# Autodesk Inventor assembly: Gear Assembly
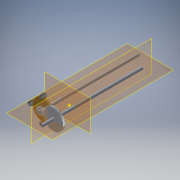
[picture p0: Inventor's stored thumbnail of the model, 180x180]
Saved by Autodesk Inventor 2016 (Build 200138000, 138)
## iProperties
Created: 2018-04-27
Part Number: Gear Assembly
Document SubType Name: Assembly
Designer: 2000083068
Author: 2000083068
## Documents named in this file (5)
- E:\Robotics\Off Season\Blannon\Gear Assembly.iam
- E:\Robotics\Off Season\Blannon\72t_Aluminum_Spur_Gear_20_DP_1_2_Hex_Bore_217-3576.ipt
- E:\Robotics\Off Season\Blannon\24t_Steel_Spur_Gear_20_DP_1_2_Hex_Bore_217-5464.ipt
- E:\Robotics\Off Season\Blannon\11t_Steel_Spur_Gear_20_DP_CIM_Motor_12t_Center_Distance_217-3107.ipt
- E:\Robotics\Off Season\Blannon\ThunderHex_Stock_18in.ipt
## Components (8 placed, 4 different names)
1. 72t_Aluminum_Spur_Gear_20_DP_1_2_Hex_Bore_217-3576:1 — Mate:1, Flush:1, Flush:2, Mate:6, Flush:4, Flush:5, Mate:12, Mate:15
2. 24t_Steel_Spur_Gear_20_DP_1_2_Hex_Bore_217-5464:1 — Mate:1, Flush:1, Flush:2, Mate:5, Mate:9, Mate:10, Mate:13
3. 72t_Aluminum_Spur_Gear_20_DP_1_2_Hex_Bore_217-3576:2 — Mate:7, Mate:8, Flush:3, Flush:4
4. 11t_Steel_Spur_Gear_20_DP_CIM_Motor_12t_Center_Distance_217-3107:1 — Mate:11, Flush:5
5. 11t_Steel_Spur_Gear_20_DP_CIM_Motor_12t_Center_Distance_217-3107:2 — Mate:5, Mate:6, Mate:14
6. 11t_Steel_Spur_Gear_20_DP_CIM_Motor_12t_Center_Distance_217-3107:3 — Mate:12, Mate:13
7. ThunderHex_Stock_18in:1 — Mate:7, Mate:8, Flush:3, Flush:6, Mate:16
8. ThunderHex_Stock_18in:2 — Mate:9, Mate:10, Mate:11, Flush:6
## Relationships (19: Mate 13, Flush 6)
- Mate:1: 72t_Aluminum_Spur_Gear_20_DP_1_2_Hex_Bore_217-3576:1 ↔ 24t_Steel_Spur_Gear_20_DP_1_2_Hex_Bore_217-5464:1
- Flush:1: 72t_Aluminum_Spur_Gear_20_DP_1_2_Hex_Bore_217-3576:1 ↔ 24t_Steel_Spur_Gear_20_DP_1_2_Hex_Bore_217-5464:1
- Flush:2: 72t_Aluminum_Spur_Gear_20_DP_1_2_Hex_Bore_217-3576:1 ↔ 24t_Steel_Spur_Gear_20_DP_1_2_Hex_Bore_217-5464:1
- Mate:5 (-42.164 mm): 24t_Steel_Spur_Gear_20_DP_1_2_Hex_Bore_217-5464:1 ↔ 11t_Steel_Spur_Gear_20_DP_CIM_Motor_12t_Center_Distance_217-3107:2
- Mate:6 (-12.7 mm): 72t_Aluminum_Spur_Gear_20_DP_1_2_Hex_Bore_217-3576:1 ↔ 11t_Steel_Spur_Gear_20_DP_CIM_Motor_12t_Center_Distance_217-3107:2
- Mate:7: 72t_Aluminum_Spur_Gear_20_DP_1_2_Hex_Bore_217-3576:2 ↔ ThunderHex_Stock_18in:1
- Mate:8: 72t_Aluminum_Spur_Gear_20_DP_1_2_Hex_Bore_217-3576:2 ↔ ThunderHex_Stock_18in:1
- Mate:9: 24t_Steel_Spur_Gear_20_DP_1_2_Hex_Bore_217-5464:1 ↔ ThunderHex_Stock_18in:2
- Mate:10: 24t_Steel_Spur_Gear_20_DP_1_2_Hex_Bore_217-5464:1 ↔ ThunderHex_Stock_18in:2
- Flush:3 (-50.8 mm): 72t_Aluminum_Spur_Gear_20_DP_1_2_Hex_Bore_217-3576:2 ↔ ThunderHex_Stock_18in:1
- Flush:4 (-12.7 mm): 72t_Aluminum_Spur_Gear_20_DP_1_2_Hex_Bore_217-3576:1 ↔ 72t_Aluminum_Spur_Gear_20_DP_1_2_Hex_Bore_217-3576:2
- Mate:11 (52.324 mm): 11t_Steel_Spur_Gear_20_DP_CIM_Motor_12t_Center_Distance_217-3107:1 ↔ ThunderHex_Stock_18in:2
- Flush:5 (5.08 mm): 72t_Aluminum_Spur_Gear_20_DP_1_2_Hex_Bore_217-3576:1 ↔ 11t_Steel_Spur_Gear_20_DP_CIM_Motor_12t_Center_Distance_217-3107:1
- Mate:12 (-12.7 mm): 72t_Aluminum_Spur_Gear_20_DP_1_2_Hex_Bore_217-3576:1 ↔ 11t_Steel_Spur_Gear_20_DP_CIM_Motor_12t_Center_Distance_217-3107:3
- Mate:13 (44.196 mm): 24t_Steel_Spur_Gear_20_DP_1_2_Hex_Bore_217-5464:1 ↔ 11t_Steel_Spur_Gear_20_DP_CIM_Motor_12t_Center_Distance_217-3107:3
- Flush:6: ThunderHex_Stock_18in:1 ↔ ThunderHex_Stock_18in:2
- Mate:14 (-38.1 mm): 11t_Steel_Spur_Gear_20_DP_CIM_Motor_12t_Center_Distance_217-3107:2
- Mate:15 (76.2 mm): 72t_Aluminum_Spur_Gear_20_DP_1_2_Hex_Bore_217-3576:1
- Mate:16: ThunderHex_Stock_18in:1
